# Autodesk Inventor assembly: Group
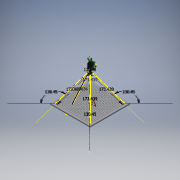
[picture p0: Inventor's stored thumbnail of the model, 180x180]
Saved by Autodesk Inventor 2018.2 (Build 222227000, 227)
## iProperties
Created: 2018-04-10
Part Number: Group
Material: Generisch
Document SubType Name: Assembly
Designer: Nick Koch
Author: Nick Koch
## Documents named in this file (7)
- C:\Users\Nick Koch\Desktop\Lehre\FHNW\Raytracing Modell\v3\Group.iam
- C:\Users\Nick Koch\Desktop\Lehre\FHNW\Raytracing Modell\v3\MiddleStick.ipt
- C:\Users\Nick Koch\Desktop\Lehre\FHNW\Raytracing Modell\v3\Screen.ipt
- C:\Users\Nick Koch\Desktop\Lehre\FHNW\Raytracing Modell\v3\Camera.ipt
- C:\Users\Nick Koch\Desktop\Lehre\FHNW\Raytracing Modell\v3\blueStick.ipt
- C:\Users\Nick Koch\Desktop\Lehre\FHNW\Raytracing Modell\v3\FOVStick.ipt
- C:\Users\Nick Koch\Desktop\Lehre\FHNW\Raytracing Modell\v3\ArrowUp.ipt
## Components (13 placed, 6 different names)
1. MiddleStick:1 — Passend:1, Passend:2, Passend:3, Passend:4, Passend:5, Passend:6, Passend:16
2. Screen:1 — Passend:1, Passend:2, Passend:3, Passend:16, Passend:21, Passend:22, Passend:23, Passend:24, Passend:25, Passend:26, Passend:27, Passend:28, Passend:29, Passend:30, Passend:31, Passend:32
3. Camera:1 — Passend:4, Passend:5, Passend:6, Passend:13, Passend:14, Passend:15, Passend:19, Passend:20, Passend:33, Passend:34, Passend:35, Passend:36, Passend:37, Passend:38, Passend:39, Passend:40, Passend:41, Passend:42, Passend:43, Passend:44, Passend:45, Passend:46, Passend:47
4. blueStick:3 — Passend:13, Passend:14, Passend:15
5. FOVStick:2 — Passend:21, Passend:22, Passend:23
6. FOVStick:3 — Passend:24, Passend:25, Passend:26
7. FOVStick:4 — Passend:27, Passend:28, Passend:29
8. FOVStick:5 — Passend:30, Passend:31, Passend:32
9. ArrowUp:1 — Passend:33, Passend:34, Passend:35
10. ArrowUp:2 — Passend:36, Passend:40, Passend:41
11. ArrowUp:3 — Passend:38, Passend:44, Passend:45
12. ArrowUp:5 — Passend:39, Passend:46, Passend:47
13. ArrowUp:6 — Passend:37, Passend:42, Passend:43
## Relationships (39: Mate 39)
- Passend:1 [Mate]: MiddleStick:1 ↔ Screen:1
- Passend:2 [Mate]: MiddleStick:1 ↔ Screen:1
- Passend:3 [Mate]: MiddleStick:1 ↔ Screen:1
- Passend:4 [Mate]: MiddleStick:1 ↔ Camera:1
- Passend:5 [Mate]: MiddleStick:1 ↔ Camera:1
- Passend:6 [Mate]: MiddleStick:1 ↔ Camera:1
- Passend:13 [Mate]: Camera:1 ↔ blueStick:3
- Passend:14 [Mate]: Camera:1 ↔ blueStick:3
- Passend:15 [Mate]: Camera:1 ↔ blueStick:3
- Passend:16 [Mate]: MiddleStick:1 ↔ Screen:1
- Passend:19 [Mate]: Camera:1
- Passend:20 [Mate]: Camera:1
- Passend:21 [Mate]: Screen:1 ↔ FOVStick:2
- Passend:22 [Mate]: Screen:1 ↔ FOVStick:2
- Passend:23 [Mate]: Screen:1 ↔ FOVStick:2
- Passend:24 [Mate]: Screen:1 ↔ FOVStick:3
- Passend:25 [Mate]: Screen:1 ↔ FOVStick:3
- Passend:26 [Mate]: Screen:1 ↔ FOVStick:3
- Passend:27 [Mate]: Screen:1 ↔ FOVStick:4
- Passend:28 [Mate]: Screen:1 ↔ FOVStick:4
- Passend:29 [Mate]: Screen:1 ↔ FOVStick:4
- Passend:30 [Mate]: Screen:1 ↔ FOVStick:5
- Passend:31 [Mate]: Screen:1 ↔ FOVStick:5
- Passend:32 [Mate]: Screen:1 ↔ FOVStick:5
- Passend:33 [Mate]: Camera:1 ↔ ArrowUp:1
- Passend:34 [Mate]: Camera:1 ↔ ArrowUp:1
- Passend:35 [Mate]: Camera:1 ↔ ArrowUp:1
- Passend:36 [Mate]: Camera:1 ↔ ArrowUp:2
- Passend:37 [Mate]: Camera:1 ↔ ArrowUp:6
- Passend:38 [Mate]: Camera:1 ↔ ArrowUp:3
- Passend:39 [Mate]: Camera:1 ↔ ArrowUp:5
- Passend:40 [Mate]: Camera:1 ↔ ArrowUp:2
- Passend:41 [Mate]: Camera:1 ↔ ArrowUp:2
- Passend:42 [Mate]: Camera:1 ↔ ArrowUp:6
- Passend:43 [Mate]: Camera:1 ↔ ArrowUp:6
- Passend:44 [Mate]: Camera:1 ↔ ArrowUp:3
- Passend:45 [Mate]: Camera:1 ↔ ArrowUp:3
- Passend:46 [Mate]: Camera:1 ↔ ArrowUp:5
- Passend:47 [Mate]: Camera:1 ↔ ArrowUp:5
